# Autodesk Inventor assembly: GFRP_T3_02
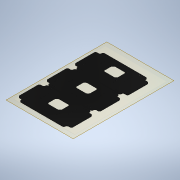
[picture p0: Inventor's stored thumbnail of the model, 180x180]
Saved by Autodesk Inventor 2022 (Build 260153000, 153)
## iProperties
Created: 2022-09-28
Part Number: GFRP_T3_02
Document SubType Name: Assembly
Designer: Masato
Author: Masato
## Documents named in this file (3)
- C:\Users\ヨコオリク\Documents\CITBrains\SUSTAINA-OP\Cam\GFRP_T3\GFRP_T3_02.iam
- C:\Users\ヨコオリク\Documents\CITBrains\SUSTAINA-OP\Cam\DisposableBoard.ipt
- C:\Users\ヨコオリク\Documents\CITBrains\SUSTAINA-OP\LowerBody\Foot\Sole_frame.ipt
## Components (4 placed, 2 different names)
1. DisposableBoard:1 — フラッシュ:1, フラッシュ:2, フラッシュ:3, フラッシュ:4, フラッシュ:5, フラッシュ:6
2. Sole_frame:1 — メイト:1, フラッシュ:5, フラッシュ:6
3. Sole_frame:2
4. Sole_frame:3
## Component patterns: (3 elements, first: Sole_frame:1)
## Relationships (7: Flush 6, Mate 1)
- フラッシュ:1 [Flush]: DisposableBoard:1
- フラッシュ:2 [Flush]: DisposableBoard:1
- フラッシュ:3 [Flush]: DisposableBoard:1
- フラッシュ:4 [Flush]: DisposableBoard:1
- メイト:1 [Mate]: Sole_frame:1
- フラッシュ:5 [Flush] (2 mm): DisposableBoard:1 ↔ Sole_frame:1
- フラッシュ:6 [Flush] (2 mm): DisposableBoard:1 ↔ Sole_frame:1
